# Autodesk Inventor assembly: mhxanh
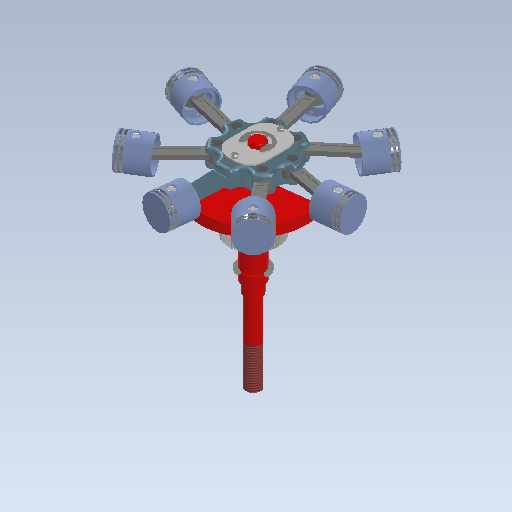
[picture p0: Inventor's stored thumbnail of the model, 512x512]
Saved by Autodesk Inventor 2021 (Build 250183000, 183)
## iProperties
Created: 2022-10-25
Part Number: mhxanh
Document SubType Name: Assembly
Designer: peris
Author: peris
## Documents named in this file (14)
- D:\Inventor\Radial_Engine\Assembly\mhxanh.iam
- D:\Inventor\Radial_Engine\Component 2.ipt
- D:\Inventor\Radial_Engine\Component 37.ipt
- D:\Inventor\Radial_Engine\Assembly\piston assembly_shunk.iam
- D:\Inventor\Radial_Engine\Component 7.ipt
- D:\Inventor\Radial_Engine\Component 16.ipt
- D:\Inventor\Radial_Engine\Component 17.ipt
- D:\Inventor\Radial_Engine\Shaft.ipt
- C:\Users\peris\OneDrive\Έγγραφα\Inventor\Content Center Files\R2021\en-US\DIN 617 SKF(2)\DIN 617 SKF - SKF NA 4900 RS.ipt
- C:\Users\peris\OneDrive\Έγγραφα\Inventor\Content Center Files\R2021\en-US\DIN 6799\DIN 6799 - 9 10.ipt
- C:\Users\peris\OneDrive\Έγγραφα\Inventor\Content Center Files\R2021\en-US\DIN 6799\DIN 6799 - 10 11.ipt
- C:\Users\peris\OneDrive\Έγγραφα\Inventor\Content Center Files\R2021\en-US\DIN 920\DIN 920 - M3 x 16.ipt
- C:\Users\peris\OneDrive\Έγγραφα\Inventor\Content Center Files\R2021\en-US\DIN EN 24 036(2)\DIN EN 24 036 - M3.ipt
- D:\Inventor\Radial_Engine\Component 6.ipt
## Components (31 placed, 13 different names)
1. Component 2:1 — Mate:1, Mate:2, Flush:1, Flush:2, Flush:3, Flush:4, Flush:5, Flush:6, Mate:22, Mate:23, Mate:36, Mate:37, Flush:7, Mate:40, Mate:41, Mate:42, Mate:47, Mate:49, Mate:52, Mate:54, Mate:58, Mate:59, Mate:60, Mate:61, Mate:62, Mate:63, Mate:74, Mate:75, Mate:76, Mate:77, Mate:80, Mate:81
2. Component 37:2 — Flush:6, Mate:62, Mate:73
3. Component 37:3 — Flush:2, Mate:63, Mate:78
4. Component 37:4 — Flush:4, Mate:59, Mate:71
5. Component 37:5 — Flush:3, Mate:58, Mate:70
6. Component 37:6 — Flush:5, Mate:60, Mate:72
7. Component 37:7 — Flush:1, Mate:61, Mate:79
8. piston assembly_shunk:1 [sub-assembly] — Mate:22, Mate:23
9. Component 7:1 — Mate:39, Mate:40, Mate:41, Mate:42, Mate:44, Mate:48, Mate:50
10. Component 16:1 — Mate:29, Mate:30, Mate:31, Mate:35
11. Component 17:1 — Mate:29, Mate:30, Mate:32, Mate:33, Mate:34, Mate:35
12. Shaft:1 — Mate:31, Mate:32, Mate:33, Mate:34, Mate:36, Mate:38, Mate:39, Mate:43, Mate:45, Mate:46
13. DIN 617 SKF- with Inner Ring - NA 49...RS SKF NA 4900 RS:1 — Mate:37, Mate:38, Flush:7
14. DIN 6799 9:1 — Mate:43, Mate:44
15. DIN 6799 10:1 — Mate:45, Mate:46
16. DIN 920 M3 x 16:1 — Mate:47, Mate:48, Mate:51
17. DIN 920 M3 x 16:2 — Mate:49, Mate:50, Mate:53
18. DIN EN 24036 M3:1 — Mate:51, Mate:52
19. DIN EN 24036 M3:2 — Mate:53, Mate:54
20. piston assembly_shunk:2 [sub-assembly] — Mate:56, Mate:57
21. piston assembly_shunk:6 [sub-assembly] — Flush:8, Mate:55
22. Component 6:1 — Mate:56, Mate:57, Mate:71, Mate:75
23. Component 6:2 — Flush:8, Mate:55, Mate:70, Mate:77
24. piston assembly_shunk:8 [sub-assembly]
25. Component 6:3 — Mate:79, Mate:80, Mate:82, Mate:83
26. Component 6:4 — Mate:78, Mate:81
27. piston assembly_shunk:9 [sub-assembly]
28. piston assembly_shunk:10 [sub-assembly]
29. Component 6:5 — Mate:72, Mate:76
30. Component 6:6 — Mate:73, Mate:74
31. piston assembly_shunk:11 [sub-assembly] — Mate:82, Mate:83
## Relationships (67: Mate 57, Flush 10)
- Mate:1: Component 2:1
- Mate:2: Component 2:1
- Flush:1: Component 2:1 ↔ Component 37:7
- Flush:2: Component 2:1 ↔ Component 37:3
- Flush:3: Component 2:1 ↔ Component 37:5
- Flush:4: Component 2:1 ↔ Component 37:4
- Flush:5: Component 2:1 ↔ Component 37:6
- Flush:6: Component 2:1 ↔ Component 37:2
- Mate:22: Component 2:1 ↔ piston assembly_shunk:1
- Mate:23 (-3.5 mm): Component 2:1 ↔ piston assembly_shunk:1
- Mate:29: Component 16:1 ↔ Component 17:1
- Mate:30: Component 16:1 ↔ Component 17:1
- Mate:31: Component 16:1 ↔ Shaft:1
- Mate:32: Component 17:1 ↔ Shaft:1
- Mate:33: Component 17:1 ↔ Shaft:1
- Mate:34: Component 17:1 ↔ Shaft:1
- Mate:35: Component 16:1 ↔ Component 17:1
- Mate:36: Component 2:1 ↔ Shaft:1
- Mate:37: Component 2:1 ↔ DIN 617 SKF- with Inner Ring - NA 49...RS SKF NA 4900 RS:1
- Mate:38: Shaft:1 ↔ DIN 617 SKF- with Inner Ring - NA 49...RS SKF NA 4900 RS:1
- Flush:7: Component 2:1 ↔ DIN 617 SKF- with Inner Ring - NA 49...RS SKF NA 4900 RS:1
- Mate:39: Component 7:1 ↔ Shaft:1
- Mate:40: Component 2:1 ↔ Component 7:1
- Mate:41: Component 2:1 ↔ Component 7:1
- Mate:42: Component 2:1 ↔ Component 7:1
- Mate:43: Shaft:1 ↔ DIN 6799 9:1
- Mate:44: Component 7:1 ↔ DIN 6799 9:1
- Mate:45: Shaft:1 ↔ DIN 6799 10:1
- Mate:46: Shaft:1 ↔ DIN 6799 10:1
- Mate:47: Component 2:1 ↔ DIN 920 M3 x 16:1
- Mate:48: Component 7:1 ↔ DIN 920 M3 x 16:1
- Mate:49: Component 2:1 ↔ DIN 920 M3 x 16:2
- Mate:50: Component 7:1 ↔ DIN 920 M3 x 16:2
- Mate:51: DIN 920 M3 x 16:1 ↔ DIN EN 24036 M3:1
- Mate:52: Component 2:1 ↔ DIN EN 24036 M3:1
- Mate:53: DIN 920 M3 x 16:2 ↔ DIN EN 24036 M3:2
- Mate:54: Component 2:1 ↔ DIN EN 24036 M3:2
- Flush:8: piston assembly_shunk:6 ↔ Component 6:2
- Mate:55: piston assembly_shunk:6 ↔ Component 6:2
- Mate:56: piston assembly_shunk:2 ↔ Component 6:1
- Mate:57: piston assembly_shunk:2 ↔ Component 6:1
- Mate:58: Component 2:1 ↔ Component 37:5
- Mate:59: Component 2:1 ↔ Component 37:4
- Mate:60: Component 2:1 ↔ Component 37:6
- Mate:61: Component 2:1 ↔ Component 37:7
- Mate:62: Component 2:1 ↔ Component 37:2
- Mate:63: Component 2:1 ↔ Component 37:3
- [Flush]: piston assembly_shunk:8 ↔ Component 6:4
- [Mate]: piston assembly_shunk:8 ↔ Component 6:4
- [Flush]: piston assembly_shunk:10 ↔ Component 6:6
- [Mate]: piston assembly_shunk:10 ↔ Component 6:6
- [Mate]: piston assembly_shunk:9 ↔ Component 6:5
- [Mate]: piston assembly_shunk:9 ↔ Component 6:5
- Mate:70: Component 37:5 ↔ Component 6:2
- Mate:71: Component 37:4 ↔ Component 6:1
- Mate:72: Component 37:6 ↔ Component 6:5
- Mate:73: Component 37:2 ↔ Component 6:6
- Mate:74: Component 2:1 ↔ Component 6:6
- Mate:75: Component 2:1 ↔ Component 6:1
- Mate:76: Component 2:1 ↔ Component 6:5
- Mate:77: Component 2:1 ↔ Component 6:2
- Mate:78: Component 37:3 ↔ Component 6:4
- Mate:79: Component 37:7 ↔ Component 6:3
- Mate:80: Component 2:1 ↔ Component 6:3
- Mate:81: Component 2:1 ↔ Component 6:4
- Mate:82: Component 6:3 ↔ piston assembly_shunk:11
- Mate:83: Component 6:3 ↔ piston assembly_shunk:11
## Named parameters: d73_d62 = 0 mm, d74_d63 = 0 mm, d76_d65 = 0 mm, d77_d62 = 0 mm, d78_d63 = 0 mm, d79_d64 = 0 mm
